# Autodesk Inventor assembly: FlipperMotorGearboxAssembly
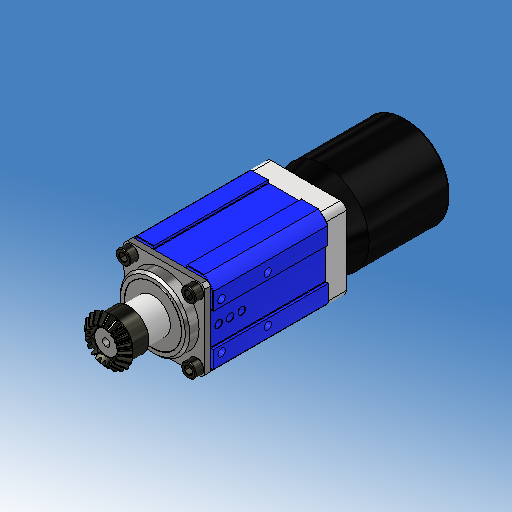
[picture p0: Inventor's stored thumbnail of the model, 512x512]
Saved by Autodesk Inventor 2025 (Build 290162000, 162)
## iProperties
Created: 2024-03-26
Part Number: FlipperMotorGearboxAssembly
Document SubType Name: Assembly
Designer: seene
Author: seene
## Documents named in this file (10)
- C:\Users\seene\OneDrive\SBRT\Robocup Rescue\Drive\v1\FlipperMotorGearboxAssembly.iam
- C:\Users\seene\OneDrive\SBRT\Robocup Rescue\Drive\v1\50XX.ipt
- C:\Users\seene\OneDrive\SBRT\Robocup Rescue\Drive\v1\FlipperH5055RoundShaft.ipt
- C:\Users\seene\OneDrive\SBRT\Robocup Rescue\Drive\v1\am-3785 - CIM Sport 16T Pinion Gear.ipt
- C:\Users\seene\OneDrive\SBRT\Robocup Rescue\Drive\v1\3 Stage HD - CIM Sport.iam
- C:\Users\seene\OneDrive\SBRT\Robocup Rescue\Drive\v1\am-3772 1.25, 20T, 500 Hex Bore.ipt
- C:\Users\seene\OneDrive\SBRT\Robocup Rescue\Drive\v1\am-3769a CIM and Falcon Sport Motor Block Short.ipt
- C:\Users\seene\OneDrive\SBRT\Robocup Rescue\Drive\v1\98541A116_External Retaining Ring.ipt
- C:\Users\seene\OneDrive\SBRT\Robocup Rescue\Drive\v1\90119A111_Low-Clearance External Retaining Rings.ipt
- C:\Users\seene\OneDrive\SBRT\Robocup Rescue\Drive\v1\SportGearbox_HexDiffGearSpacer.ipt
## Components (10 placed, 9 different names)
1. 50XX:1 — Mate:1, Mate:2, Mate:17, Mate:18, Mate:19
2. FlipperH5055RoundShaft:1 — Mate:1, Mate:2, Mate:3, Mate:23, Mate:26, Mate:27, Mate:28, Mate:29, Mate:30, Mate:31
3. am-3785 - CIM Sport 16T Pinion Gear:1 — Mate:3, Mate:23
4. 3 Stage HD - CIM Sport:1 [sub-assembly] — Mate:14, Mate:15, Mate:16, Mate:20, Mate:21, Mate:22, Mate:33, Mate:34, Flush:1
5. am-3772 1.25, 20T, 500 Hex Bore:1 — Mate:14, Mate:15, Mate:16, Mate:32
6. am-3769a CIM and Falcon Sport Motor Block Short:1 — Mate:17, Mate:18, Mate:19, Mate:20, Mate:21, Mate:22
7. 98541A116_External Retaining Ring:1 — Mate:26, Mate:27
8. 90119A111_Low-Clearance External Retaining Rings:1 — Mate:28, Mate:29
9. 90119A111_Low-Clearance External Retaining Rings:2 — Mate:30, Mate:31
10. SportGearbox_HexDiffGearSpacer:1 — Mate:32, Mate:33, Mate:34
## Relationships (23: Mate 22, Flush 1)
- Mate:1: 50XX:1 ↔ FlipperH5055RoundShaft:1
- Mate:2: 50XX:1 ↔ FlipperH5055RoundShaft:1
- Mate:3: FlipperH5055RoundShaft:1 ↔ am-3785 - CIM Sport 16T Pinion Gear:1
- Mate:14: 3 Stage HD - CIM Sport:1 ↔ am-3772 1.25, 20T, 500 Hex Bore:1
- Mate:15: 3 Stage HD - CIM Sport:1 ↔ am-3772 1.25, 20T, 500 Hex Bore:1
- Mate:16 (13.0302 mm): 3 Stage HD - CIM Sport:1 ↔ am-3772 1.25, 20T, 500 Hex Bore:1
- Mate:17: 50XX:1 ↔ am-3769a CIM and Falcon Sport Motor Block Short:1
- Mate:18: 50XX:1 ↔ am-3769a CIM and Falcon Sport Motor Block Short:1
- Mate:19: 50XX:1 ↔ am-3769a CIM and Falcon Sport Motor Block Short:1
- Mate:20: 3 Stage HD - CIM Sport:1 ↔ am-3769a CIM and Falcon Sport Motor Block Short:1
- Mate:21: 3 Stage HD - CIM Sport:1 ↔ am-3769a CIM and Falcon Sport Motor Block Short:1
- Mate:22: 3 Stage HD - CIM Sport:1 ↔ am-3769a CIM and Falcon Sport Motor Block Short:1
- Mate:23 (0.2 mm): FlipperH5055RoundShaft:1 ↔ am-3785 - CIM Sport 16T Pinion Gear:1
- Mate:26: FlipperH5055RoundShaft:1 ↔ 98541A116_External Retaining Ring:1
- Mate:27: FlipperH5055RoundShaft:1 ↔ 98541A116_External Retaining Ring:1
- Mate:28: FlipperH5055RoundShaft:1 ↔ 90119A111_Low-Clearance External Retaining Rings:1
- Mate:29: FlipperH5055RoundShaft:1 ↔ 90119A111_Low-Clearance External Retaining Rings:1
- Mate:30: FlipperH5055RoundShaft:1 ↔ 90119A111_Low-Clearance External Retaining Rings:2
- Mate:31: FlipperH5055RoundShaft:1 ↔ 90119A111_Low-Clearance External Retaining Rings:2
- Mate:32: am-3772 1.25, 20T, 500 Hex Bore:1 ↔ SportGearbox_HexDiffGearSpacer:1
- Mate:33: 3 Stage HD - CIM Sport:1 ↔ SportGearbox_HexDiffGearSpacer:1
- Mate:34: 3 Stage HD - CIM Sport:1 ↔ SportGearbox_HexDiffGearSpacer:1
- Flush:1 (0.9189 mm): 3 Stage HD - CIM Sport:1
